# Autodesk Inventor assembly: 00-05-RubberFoot
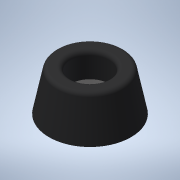
[picture p0: Inventor's stored thumbnail of the model, 180x180]
Saved by Autodesk Inventor 2022 (Build 260153000, 153)
## iProperties
Created: 2019-05-31
Part Number: 00-05-RubberFoot
Material: Generisch
Document SubType Name: Assembly
Designer: denni
Author: denni
## Documents named in this file (3)
- D:\Inventor\3D Printer\00-PurchasedParts\00-05-RubberFeet\00-05-RubberFoot.iam
- D:\Inventor\3D Printer\00-PurchasedParts\00-05-RubberFeet\00-05-001-Rubber.ipt
- D:\Inventor\3D Printer\00-PurchasedParts\00-05-RubberFeet\00-05-002-MetalDisk.ipt
## Components (2 placed, 2 different names)
1. 00-05-001-Rubber:1 — Passend:1, Passend:2, Fluchtend:1, Fluchtend:2, Fluchtend:3
2. 00-05-002-MetalDisk:1 — Passend:1, Passend:2
## Relationships (5: Flush 3, Mate 2)
- Passend:1 [Mate]: 00-05-001-Rubber:1 ↔ 00-05-002-MetalDisk:1
- Passend:2 [Mate]: 00-05-001-Rubber:1 ↔ 00-05-002-MetalDisk:1
- Fluchtend:1 [Flush]: 00-05-001-Rubber:1
- Fluchtend:2 [Flush]: 00-05-001-Rubber:1
- Fluchtend:3 [Flush]: 00-05-001-Rubber:1
